# Autodesk Inventor assembly: wafel_rev2
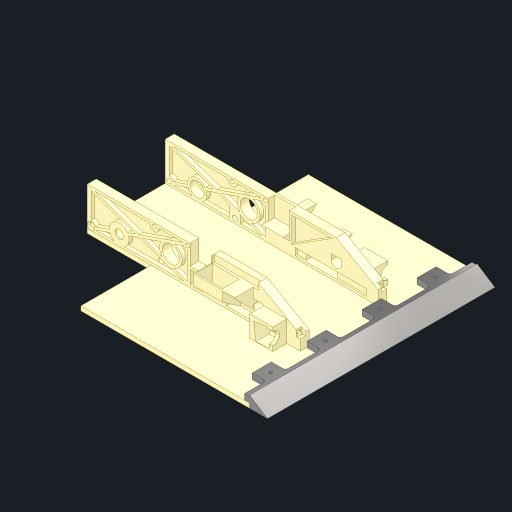
[picture p0: Inventor's stored thumbnail of the model, 512x512]
Saved by Autodesk Inventor 2023 (Build 270158000, 158)
## iProperties
Created: 2024-04-29
Part Number: wafel_rev2
Document SubType Name: Assembly
Designer: szymo
Mass: 1047.95 g
Surface Area: 2382.84 cm^2
Volume: 542.867 cm^3
Density: 1.93041 g/cm^3
Author: szymo
## Documents named in this file (23)
- C:\zRozne\roboilo\robots\codename wafel - australia\3d_parts\rev2\wafel_rev2.iam
- C:\zRozne\roboilo\robots\codename wafel - australia\3d_parts\rev2\plog.ipt
- C:\zRozne\roboilo\robots\codename wafel - australia\3d_parts\rev2\smolgear_shaft.ipt
- C:\zRozne\roboilo\robots\codename wafel - australia\3d_parts\rev2\smolLipo.ipt
- C:\zRozne\roboilo\robots\codename wafel - australia\3d_parts\rev2\stack.iam
- C:\zRozne\roboilo\robots\codename wafel - australia\3d_parts\rev2\Switch.ipt
- C:\zRozne\roboilo\robots\codename wafel - australia\3d_parts\rev2\TFMiniS.ipt
- C:\zRozne\roboilo\robots\codename wafel - australia\3d_parts\rev2\wheel_axle.iam
- C:\zRozne\roboilo\robots\codename wafel - australia\3d_parts\rev2\KTIR-Board.ipt
- C:\zRozne\roboilo\robots\codename wafel - australia\3d_parts\rev2\lipo3s650.ipt
- C:\zRozne\roboilo\robots\codename wafel - australia\3d_parts\rev2\Design Accelerator\smolGear.iam
- C:\zRozne\roboilo\robots\codename wafel - australia\3d_parts\rev2\motor_w_gear.iam
- C:\zRozne\roboilo\robots\codename wafel - australia\3d_parts\rev2\base.ipt
- C:\zRozne\roboilo\robots\codename wafel - australia\3d_parts\rev2\wheel.ipt
- C:\zRozne\roboilo\robots\codename wafel - australia\3d_parts\rev2\right_hold.ipt
- C:\zRozne\roboilo\robots\codename wafel - australia\3d_parts\rev2\left_hold.ipt
- C:\zRozne\roboilo\robots\codename wafel - australia\3d_parts\rev2\front_motur_holder.ipt
- C:\zRozne\roboilo\robots\codename wafel - australia\3d_parts\rev2\front_motur_holder_MIR.ipt
- C:\zRozne\roboilo\robots\codename wafel - australia\3d_parts\rev2\right_gear_holder.ipt
- C:\zRozne\roboilo\robots\codename wafel - australia\3d_parts\rev2\right_gear_holder_MIR.ipt
- C:\zRozne\roboilo\robots\codename wafel - australia\3d_parts\rev2\interface_board.ipt
- C:\zRozne\roboilo\robots\codename wafel - australia\3d_parts\rev2\back.ipt
- C:\zRozne\roboilo\robots\codename wafel - australia\3d_parts\rev2\oled.ipt
## Components (29 placed, 22 different names)
1. base:1 — Flush:1, Mate:2, Tangent:1, Angle:1, Tangent:2, Mate:5, Angle:2, Tangent:6, Flush:7, Flush:8, Tangent:7, Mate:7, Flush:9, Flush:10, Flush:17, Flush:21, Flush:22, Mate:14
2. plog:1 — Flush:1, Mate:2, Mate:9, Angle:3, Angle:4
3. right_hold:1 — Flush:10, Flush:11, Flush:20, Mate:13, Mate:15, Mate:16, Mate:21, Mate:22, Flush:24, Mate:23, Mate:24, Flush:26, Flush:27, Flush:30, Flush:31, Flush:32, Flush:34, Symmetry:18, Symmetry:19, Symmetry:20
4. left_hold:1 — Mate:17, Mate:19, Flush:23, Symmetry:18, Symmetry:19, Symmetry:20, Flush:35, Flush:36
5. right_gear_holder_MIR:1
6. right_gear_holder:1 — Flush:17, Flush:20
7. front_motur_holder_MIR:1 — Mate:20
8. front_motur_holder:1
9. TFMiniS:1 — Mate:14, Angle:3, Mate:15, Angle:4, Mate:16, Symmetry:15, Symmetry:16, Symmetry:17, Flush:30, Flush:31, Flush:32, Flush:34
10. wheel_axle:1 [sub-assembly] — Flush:2, Flush:3, Mate:3, Mate:4, Tangent:1, Tangent:5, Symmetry:3, Symmetry:4, Mate:6
11. smolGear:1 [sub-assembly] — Flush:3, Tangent:4, Tangent:5, Symmetry:5, Symmetry:12, Mate:12
12. wheel:1 — Mate:3, Mate:4, Angle:1, Tangent:6, Symmetry:1, Symmetry:2
13. motor_w_gear:1 [sub-assembly] — Flush:2, Tangent:2, Tangent:4, Angle:2, Symmetry:9, Symmetry:10, Symmetry:11, Tangent:7, Tangent:8
14. motor_w_gear:2 [sub-assembly] — Symmetry:9, Symmetry:10, Symmetry:11
15. wheel_axle:2 [sub-assembly] — Symmetry:3, Symmetry:4
16. TFMiniS:2 — Symmetry:15, Symmetry:16, Symmetry:17
17. smolGear:2 [sub-assembly] — Symmetry:5, Symmetry:12
18. wheel:2 — Symmetry:1, Symmetry:2
19. lipo3s650:1 — Mate:5, Flush:7, Flush:8, Mate:6
20. smolLipo:1 — Flush:11, Tangent:8, Mate:17
21. smolgear_shaft:1 — Symmetry:13, Symmetry:14
22. smolgear_shaft:2 — Mate:12, Mate:13, Symmetry:13, Symmetry:14
23. stack:1 [sub-assembly] — Mate:7, Flush:9, Mate:9
24. Switch:1 — Flush:25, Mate:23, Mate:24
25. KTIR-Board:1
26. KTIR-Board:2
27. interface_board:1 — Mate:19, Flush:23, Mate:20, Flush:35, Flush:36
28. back:1 — Flush:21, Flush:22
29. oled:1 — Mate:21, Mate:22, Flush:24, Flush:25, Flush:26, Flush:27
## Relationships (70: Flush 23, Mate 19, Symmetry 17, Tangent 7, Angle 4)
- Flush:1: base:1 ↔ plog:1
- Mate:2: base:1 ↔ plog:1
- Flush:2: wheel_axle:1 ↔ motor_w_gear:1
- Flush:3: wheel_axle:1 ↔ smolGear:1
- Mate:3: wheel_axle:1 ↔ wheel:1
- Mate:4 (2 mm): wheel_axle:1 ↔ wheel:1
- Tangent:1 (3 mm): base:1 ↔ wheel_axle:1
- Angle:1 (0 deg): base:1 ↔ wheel:1
- Tangent:2 (1 mm): base:1 ↔ motor_w_gear:1
- Tangent:4: smolGear:1 ↔ motor_w_gear:1
- Tangent:5: wheel_axle:1 ↔ smolGear:1
- Mate:5: base:1 ↔ lipo3s650:1
- Angle:2 (0 deg): base:1 ↔ motor_w_gear:1
- Tangent:6 (2.5 mm): base:1 ↔ wheel:1
- Symmetry:1: wheel:1 ↔ wheel:2
- Symmetry:2: wheel:1 ↔ wheel:2
- Symmetry:3: wheel_axle:1 ↔ wheel_axle:2
- Symmetry:4: wheel_axle:1 ↔ wheel_axle:2
- Symmetry:5: smolGear:1 ↔ smolGear:2
- Symmetry:9: motor_w_gear:1 ↔ motor_w_gear:2
- Symmetry:10: motor_w_gear:1 ↔ motor_w_gear:2
- Symmetry:11: motor_w_gear:1 ↔ motor_w_gear:2
- Symmetry:12: smolGear:1 ↔ smolGear:2
- Flush:7 (79 mm): base:1 ↔ lipo3s650:1
- Flush:8: base:1 ↔ lipo3s650:1
- Tangent:7 (1 mm): base:1 ↔ motor_w_gear:1
- Mate:6 (1 mm): wheel_axle:1 ↔ lipo3s650:1
- Mate:7 (2 mm): base:1 ↔ stack:1
- Flush:9 (61.5 mm): base:1 ↔ stack:1
- Flush:10: base:1 ↔ right_hold:1
- Mate:9 (10 mm): plog:1 ↔ stack:1
- Flush:11: right_hold:1 ↔ smolLipo:1
- Tangent:8 (1 mm): motor_w_gear:1 ↔ smolLipo:1
- Flush:17: base:1 ↔ right_gear_holder:1
- Flush:20 (16 mm): right_hold:1 ↔ right_gear_holder:1
- Mate:12: smolGear:1 ↔ smolgear_shaft:2
- Mate:13: right_hold:1 ↔ smolgear_shaft:2
- Symmetry:13: smolgear_shaft:1 ↔ smolgear_shaft:2
- Symmetry:14: smolgear_shaft:1 ↔ smolgear_shaft:2
- Flush:21: base:1 ↔ back:1
- Flush:22: base:1 ↔ back:1
- Mate:14: base:1 ↔ TFMiniS:1
- Angle:3 (353.5 deg): plog:1 ↔ TFMiniS:1
- Mate:15: right_hold:1 ↔ TFMiniS:1
- Angle:4 (0 deg): plog:1 ↔ TFMiniS:1
- Mate:16 (-13 mm): right_hold:1 ↔ TFMiniS:1
- Symmetry:15: TFMiniS:1 ↔ TFMiniS:2
- Symmetry:16: TFMiniS:1 ↔ TFMiniS:2
- Symmetry:17: TFMiniS:1 ↔ TFMiniS:2
- Mate:17: left_hold:1 ↔ smolLipo:1
- Mate:19: left_hold:1 ↔ interface_board:1
- Flush:23 (-5 mm): left_hold:1 ↔ interface_board:1
- Mate:20 (5 mm): front_motur_holder_MIR:1 ↔ interface_board:1
- Mate:21: right_hold:1 ↔ oled:1
- Mate:22: right_hold:1 ↔ oled:1
- Flush:24 (-3 mm): right_hold:1 ↔ oled:1
- Flush:25: Switch:1 ↔ oled:1
- Mate:23 (0.15 mm): right_hold:1 ↔ Switch:1
- Mate:24: right_hold:1 ↔ Switch:1
- Flush:26: right_hold:1 ↔ oled:1
- Flush:27: right_hold:1 ↔ oled:1
- Flush:30: right_hold:1 ↔ TFMiniS:1
- Flush:31: right_hold:1 ↔ TFMiniS:1
- Flush:32: right_hold:1 ↔ TFMiniS:1
- Flush:34: right_hold:1 ↔ TFMiniS:1
- Symmetry:18: right_hold:1 ↔ left_hold:1
- Symmetry:19: right_hold:1 ↔ left_hold:1
- Symmetry:20: right_hold:1 ↔ left_hold:1
- Flush:35: left_hold:1 ↔ interface_board:1
- Flush:36: left_hold:1 ↔ interface_board:1
